# Autodesk Inventor assembly: TPU UNIBODY Assembly 9
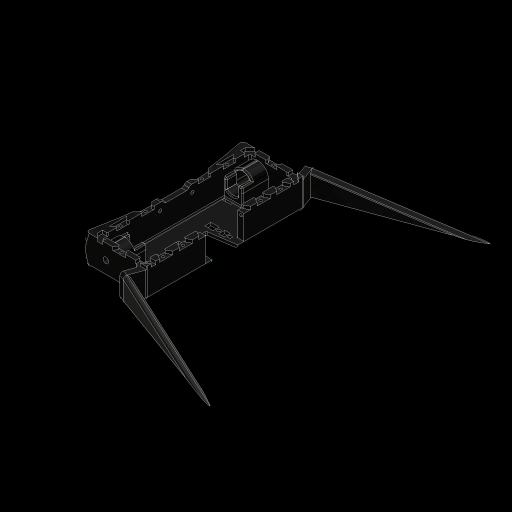
[picture p0: Inventor's stored thumbnail of the model, 512x512]
Saved by Autodesk Inventor 2023 (Build 270158000, 158)
## iProperties
Created: 2022-02-23
Part Number: TPU UNIBODY Assembly 9
Document SubType Name: Assembly
Designer: tandu
Mass: 411.334 g
Surface Area: 1467.6 cm^2
Volume: 273.151 cm^3
Density: 1.50589 g/cm^3
Author: tandu
## Documents named in this file (9)
- C:\Users\tandu\Documents\GrabCAD\Insomnia 2020\Versions\11 Wheel Guards and AR500 Blade\TPU UNIBODY Assembly 9.iam
- C:\Users\tandu\Documents\GrabCAD\Insomnia 2020\Versions\11 Wheel Guards and AR500 Blade\EMax RS2205 v1.ipt
- C:\Users\tandu\Documents\GrabCAD\Insomnia 2020\Versions\11 Wheel Guards and AR500 Blade\TPU 22 Chassis.ipt
- C:\Users\tandu\Documents\GrabCAD\Insomnia 2020\Versions\11 Wheel Guards and AR500 Blade\UHMWMotorUpright.ipt
- C:\Users\tandu\Documents\GrabCAD\Insomnia 2020\Versions\11 Wheel Guards and AR500 Blade\UHMWBearingUpright.ipt
- C:\Users\tandu\Documents\GrabCAD\Insomnia 2020\Versions\11 Wheel Guards and AR500 Blade\WedgeUHMWPiece.ipt
- C:\Users\tandu\Documents\GrabCAD\Insomnia 2020\Versions\11 Wheel Guards and AR500 Blade\WedgeUHMWPiece_MIR.ipt
- E:\Users\tandu\Documents\GrabCAD\Insomnia 2020\Versions\9 Comically Large Weapon 9 28 22\FT Clamping Weapon\Viper-V-Spinner-Add-On.iam
- E:\Users\tandu\Documents\GrabCAD\Insomnia 2020\Versions\9 Comically Large Weapon 9 28 22\TPUWeapon\TPUWeaponAssembly.iam
## Components (9 placed, 8 different names)
1. TPU 22 Chassis:1 — Insert:11, Insert:12, Insert:13, Insert:14, Insert:18, Insert:19, Insert:20, Insert:21, Insert:22, Insert:23
2. UHMWMotorUpright:1 — Insert:11, Insert:12, Insert:15, Insert:16, Symmetry:1
3. UHMWBearingUpright:1 — Insert:13, Insert:14, Symmetry:1
4. EMax RS2205 v1:1 — Insert:15, Insert:16
5. WedgeUHMWPiece:1 — Insert:20, Insert:21
6. WedgeUHMWPiece:2 — Insert:18, Insert:19, Mate:8
7. WedgePiece_MIR:1 — Mate:9, Insert:22, Insert:23
8. Viper-V-Spinner-Add-On:1 [sub-assembly] — Flush:1
9. TPUWeaponAssembly:1 [sub-assembly]
## Relationships (17: Insert 12, Mate 3, Symmetry 1, Flush 1)
- Insert:11: TPU 22 Chassis:1 ↔ UHMWMotorUpright:1
- Insert:12: TPU 22 Chassis:1 ↔ UHMWMotorUpright:1
- Insert:13: TPU 22 Chassis:1 ↔ UHMWBearingUpright:1
- Insert:14: TPU 22 Chassis:1 ↔ UHMWBearingUpright:1
- Insert:15: UHMWMotorUpright:1 ↔ EMax RS2205 v1:1
- Insert:16: UHMWMotorUpright:1 ↔ EMax RS2205 v1:1
- Insert:18: TPU 22 Chassis:1 ↔ WedgeUHMWPiece:2
- Insert:19: TPU 22 Chassis:1 ↔ WedgeUHMWPiece:2
- Insert:20: TPU 22 Chassis:1 ↔ WedgeUHMWPiece:1
- Insert:21: TPU 22 Chassis:1 ↔ WedgeUHMWPiece:1
- Symmetry:1: UHMWMotorUpright:1 ↔ UHMWBearingUpright:1
- Mate:8: WedgeUHMWPiece:2
- Mate:9: WedgePiece_MIR:1
- Mate:10
- Flush:1: Viper-V-Spinner-Add-On:1
- Insert:22: TPU 22 Chassis:1 ↔ WedgePiece_MIR:1
- Insert:23: TPU 22 Chassis:1 ↔ WedgePiece_MIR:1
